# Autodesk Inventor assembly: outside-join-no-hole
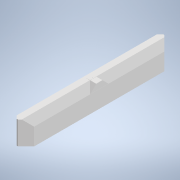
[picture p0: Inventor's stored thumbnail of the model, 180x180]
Saved by Autodesk Inventor 2021 (Build 250183000, 183)
## iProperties
Created: 2020-12-10
Part Number: outside-join-no-hole
Document SubType Name: Assembly
Designer: Luke Kamols
Author: Luke Kamols
## Documents named in this file (3)
- C:\Users\Luke Kamols\OneDrive\Documents\Other\Chess\outside-join-no-hole.iam
- C:\Users\Luke Kamols\OneDrive\Documents\Other\Chess\outside-join-half.ipt
- C:\Users\Luke Kamols\OneDrive\Documents\Other\Chess\middle-join.ipt
## Components (3 placed, 2 different names)
1. outside-join-half:1 — Mate:1, Flush:1, Flush:2, Flush:5
2. outside-join-half:2 — Mate:1, Flush:1, Flush:2, Flush:3, Flush:4
3. middle-join:1 — Flush:3, Flush:4, Flush:5
## Relationships (6: Flush 5, Mate 1)
- Mate:1: outside-join-half:1 ↔ outside-join-half:2
- Flush:1: outside-join-half:1 ↔ outside-join-half:2
- Flush:2: outside-join-half:1 ↔ outside-join-half:2
- Flush:3: outside-join-half:2 ↔ middle-join:1
- Flush:4: outside-join-half:2 ↔ middle-join:1
- Flush:5 (6 mm): outside-join-half:1 ↔ middle-join:1
